# Autodesk Inventor assembly: Spindle_Block_ASM
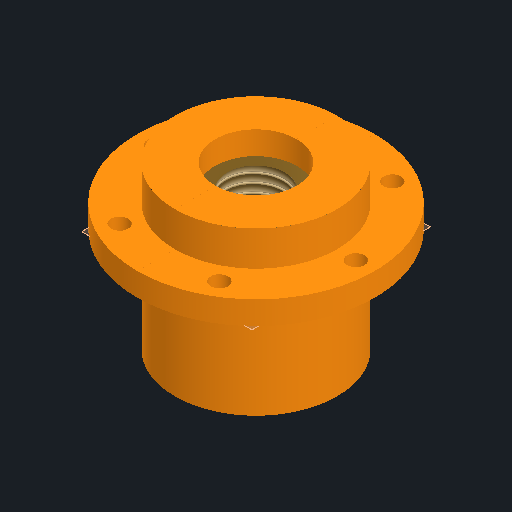
[picture p0: Inventor's stored thumbnail of the model, 512x512]
Saved by Autodesk Inventor 2024.1 (Build 281209000, 209)
## iProperties
Created: 2023-08-04
Part Number: Spindle_Block_ASM
Document SubType Name: Assembly
Designer: jaege
Author: jaege
## Documents named in this file (3)
- C:\Users\jaege\VUB\Schakel_Ind_Elo\Year_1_Both\BA_Thesis\3D_Files\Lift_V2\Spindle_Block_ASM.iam
- C:\Users\jaege\VUB\Schakel_Ind_Elo\Year_1_Both\BA_Thesis\3D_Files\Lift_V2\SpindleBlock.ipt
- C:\Users\jaege\VUB\Schakel_Ind_Elo\Year_1_Both\BA_Thesis\3D_Files\Lift_V2\Spindle_Block_Holder.ipt
## Components (3 placed, 2 different names)
1. SpindleBlock:1
2. Spindle_Block_Holder:1
3. Spindle_Block_Holder:2
## Relationships (5: Mate 5)
- [Mate]: SpindleBlock:1 ↔ Spindle_Block_Holder:1
- [Mate]: SpindleBlock:1 ↔ Spindle_Block_Holder:1
- [Mate]: Spindle_Block_Holder:1 ↔ Spindle_Block_Holder:2
- [Mate]: SpindleBlock:1 ↔ Spindle_Block_Holder:2
- [Mate]: SpindleBlock:1 ↔ Spindle_Block_Holder:2
